# Autodesk Inventor assembly: Gear_Test_4
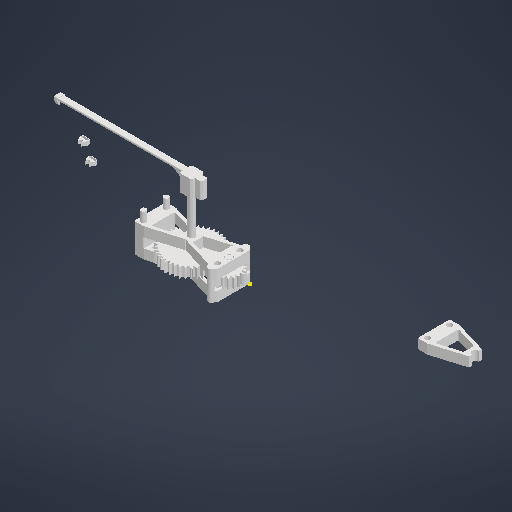
[picture p0: Inventor's stored thumbnail of the model, 512x512]
Saved by Autodesk Inventor 2026.2 (Build 302298000, 298)
## iProperties
Created: 2025-12-19
Part Number: Gear_Test_4
Document SubType Name: Assembly
Designer: Cobble
Author: Cobble
## Documents named in this file (12)
- D:\CAD\Gear_Test_4.iam
- D:\CAD\36mm_18N_Gear.ipt
- D:\CAD\Rod_support_1.ipt
- D:\CAD\8x60mm_Rod.ipt
- D:\CAD\10x120mm_Rod.ipt
- D:\CAD\Support_Seperator.ipt
- D:\CAD\80mm_40N_Gear.ipt
- D:\CAD\Rod_support_2.ipt
- D:\CAD\10x45mm_Rod.ipt
- D:\CAD\Rod_support_2.1.ipt
- D:\CAD\Turret_Holder_2_test.ipt
- D:\CAD\Turret_Holder_2_test_pt2.ipt
## Components (16 placed, 11 different names)
1. 36mm_18N_Gear:1 — Rotation:1, Insert:27
2. Rod_support_1:3 — Insert:16, Insert:17, Mate:5, Mate:6
3. Rod_support_1:4
4. 8x60mm_Rod:3 — Insert:24
5. 8x60mm_Rod:4 — Insert:23
6. 10x120mm_Rod:1 — Rotation:3, Insert:25, Insert:31
7. Support_Seperator:2 — Insert:16, Insert:17, Mate:1, Mate:2
8. 80mm_40N_Gear:1 — Rotation:1, Rotation:3, Insert:30
9. Rod_support_2:1 — Insert:21, Insert:22, Mate:5, Mate:6
10. 10x45mm_Rod:1 — Insert:26
11. Rod_support_2.1:1 — Insert:21, Insert:22, Insert:26, Insert:27
12. Rod_support_1:5 — Mate:1, Mate:2, Insert:23, Insert:24, Insert:25, Insert:30
13. Turret_Holder_2_test:1 — Insert:31, Angle:1, Angle:2
14. Turret_Holder_2_test_pt2:1
15. Turret_Holder_2_test_pt2:2 — Angle:1, Angle:2
16. Turret_Holder_2_test_pt2:3
## Relationships (19: Insert 11, Mate 4, RelateRotation 2, Angle 2)
- Rotation:1 [RelateRotation] (2.2222 ul): 36mm_18N_Gear:1 ↔ 80mm_40N_Gear:1
- Insert:16: Rod_support_1:3 ↔ Support_Seperator:2
- Insert:17: Rod_support_1:3 ↔ Support_Seperator:2
- Rotation:3 [RelateRotation] (1 ul): 10x120mm_Rod:1 ↔ 80mm_40N_Gear:1
- Insert:21: Rod_support_2:1 ↔ Rod_support_2.1:1
- Insert:22: Rod_support_2:1 ↔ Rod_support_2.1:1
- Mate:1: Support_Seperator:2 ↔ Rod_support_1:5
- Mate:2: Support_Seperator:2 ↔ Rod_support_1:5
- Insert:23: 8x60mm_Rod:4 ↔ Rod_support_1:5
- Insert:24: 8x60mm_Rod:3 ↔ Rod_support_1:5
- Mate:5: Rod_support_1:3 ↔ Rod_support_2:1
- Mate:6: Rod_support_1:3 ↔ Rod_support_2:1
- Insert:25: 10x120mm_Rod:1 ↔ Rod_support_1:5
- Insert:26: 10x45mm_Rod:1 ↔ Rod_support_2.1:1
- Insert:27: 36mm_18N_Gear:1 ↔ Rod_support_2.1:1
- Insert:30: 80mm_40N_Gear:1 ↔ Rod_support_1:5
- Insert:31: 10x120mm_Rod:1 ↔ Turret_Holder_2_test:1
- Angle:1 (0 deg): Turret_Holder_2_test:1 ↔ Turret_Holder_2_test_pt2:2
- Angle:2 (360 deg): Turret_Holder_2_test:1 ↔ Turret_Holder_2_test_pt2:2
